# Autodesk Inventor assembly: Chassis assembly
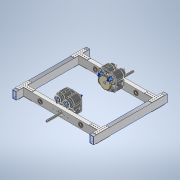
[picture p0: Inventor's stored thumbnail of the model, 180x180]
Saved by Autodesk Inventor 2022 (Build 260153000, 153)
## iProperties
Created: 2022-11-14
Part Number: Chassis assembly
Document SubType Name: Assembly
Designer: s135320
Author: s135320
## Documents named in this file (6)
- D:\Chassis assembly.iam
- D:\Chassis side 1.ipt
- D:\Chassis side 2.ipt
- D:\STEP Files\Hardware\Gussets\TTB T Gusset\TTB-00012_T-Gusset.ipt
- D:\STEP Files\Bearings\1-2inch Hex Bering\217-3875-STEP-20140818.ipt
- D:\STEP Files\Gearboxes\WCP SS Flipped Gearbox\WCP-0235.iam
## Components (22 placed, 5 different names)
1. Chassis side 1:1 — Mate:8, Mate:9, Flush:3, Mate:10, Mate:11, Flush:4, Mate:22, Mate:29, Mate:30, Mate:31, Mate:32, Mate:37, Mate:38, Mate:39, Mate:40, Mate:41, Mate:42, Mate:45
2. Chassis side 1:2 — Mate:1, Mate:2, Mate:3, Mate:14, Mate:15, Flush:6, Mate:16, Mate:17, Flush:7, Mate:20, Mate:25, Mate:26, Mate:27, Mate:28, Mate:33, Mate:34, Mate:35, Mate:36, Mate:43, Mate:44, Mate:46
3. Chassis side 2:1 — Mate:12, Mate:13, Flush:5, Mate:21, Flush:9, Mate:23, Mate:24
4. Chassis side 2:2 — Mate:4, Mate:5, Flush:1, Mate:6, Mate:7, Flush:2, Mate:18, Mate:19, Flush:8
5. TTB-00012_T-Gusset:1 — Mate:14, Mate:15, Flush:6
6. TTB-00012_T-Gusset:2 — Mate:1, Mate:2, Mate:3, Mate:4, Mate:5, Flush:1
7. TTB-00012_T-Gusset:3 — Mate:22, Mate:23, Mate:24
8. TTB-00012_T-Gusset:4 — Mate:16, Mate:17, Flush:7
9. TTB-00012_T-Gusset:5 — Mate:20, Mate:21, Flush:9
10. TTB-00012_T-Gusset:6 — Mate:6, Mate:7, Flush:2, Mate:8, Mate:9, Flush:3
11. TTB-00012_T-Gusset:7 — Mate:10, Mate:11, Flush:4, Mate:12, Mate:13, Flush:5
12. TTB-00012_T-Gusset:8 — Mate:18, Mate:19, Flush:8
13. 217-3875-STEP-20140818:3 — Mate:37, Mate:38
14. 217-3875-STEP-20140818:4 — Mate:29, Mate:30
15. 217-3875-STEP-20140818:5 — Mate:39, Mate:40
16. 217-3875-STEP-20140818:6 — Mate:35, Mate:36
17. 217-3875-STEP-20140818:8 — Mate:33, Mate:34
18. 217-3875-STEP-20140818:9 — Mate:31, Mate:32
19. 217-3875-STEP-20140818:11 — Mate:27, Mate:28
20. 217-3875-STEP-20140818:12 — Mate:25, Mate:26
21. WCP-0235:1 [sub-assembly] — Mate:43, Mate:44, Mate:46
22. WCP-0235:2 [sub-assembly] — Mate:41, Mate:42, Mate:45
## Relationships (55: Mate 46, Flush 9)
- Mate:1: Chassis side 1:2 ↔ TTB-00012_T-Gusset:2
- Mate:2: Chassis side 1:2 ↔ TTB-00012_T-Gusset:2
- Mate:3: Chassis side 1:2 ↔ TTB-00012_T-Gusset:2
- Mate:4: Chassis side 2:2 ↔ TTB-00012_T-Gusset:2
- Mate:5: Chassis side 2:2 ↔ TTB-00012_T-Gusset:2
- Flush:1: Chassis side 2:2 ↔ TTB-00012_T-Gusset:2
- Mate:6: Chassis side 2:2 ↔ TTB-00012_T-Gusset:6
- Mate:7: Chassis side 2:2 ↔ TTB-00012_T-Gusset:6
- Flush:2: Chassis side 2:2 ↔ TTB-00012_T-Gusset:6
- Mate:8: Chassis side 1:1 ↔ TTB-00012_T-Gusset:6
- Mate:9: Chassis side 1:1 ↔ TTB-00012_T-Gusset:6
- Flush:3: Chassis side 1:1 ↔ TTB-00012_T-Gusset:6
- Mate:10: Chassis side 1:1 ↔ TTB-00012_T-Gusset:7
- Mate:11: Chassis side 1:1 ↔ TTB-00012_T-Gusset:7
- Flush:4: Chassis side 1:1 ↔ TTB-00012_T-Gusset:7
- Mate:12: Chassis side 2:1 ↔ TTB-00012_T-Gusset:7
- Mate:13: Chassis side 2:1 ↔ TTB-00012_T-Gusset:7
- Flush:5: Chassis side 2:1 ↔ TTB-00012_T-Gusset:7
- Mate:14: Chassis side 1:2 ↔ TTB-00012_T-Gusset:1
- Mate:15: Chassis side 1:2 ↔ TTB-00012_T-Gusset:1
- Flush:6: Chassis side 1:2 ↔ TTB-00012_T-Gusset:1
- Mate:16: Chassis side 1:2 ↔ TTB-00012_T-Gusset:4
- Mate:17: Chassis side 1:2 ↔ TTB-00012_T-Gusset:4
- Flush:7: Chassis side 1:2 ↔ TTB-00012_T-Gusset:4
- Mate:18: Chassis side 2:2 ↔ TTB-00012_T-Gusset:8
- Mate:19: Chassis side 2:2 ↔ TTB-00012_T-Gusset:8
- Flush:8: Chassis side 2:2 ↔ TTB-00012_T-Gusset:8
- Mate:20: Chassis side 1:2 ↔ TTB-00012_T-Gusset:5
- Mate:21: Chassis side 2:1 ↔ TTB-00012_T-Gusset:5
- Flush:9: Chassis side 2:1 ↔ TTB-00012_T-Gusset:5
- Mate:22: Chassis side 1:1 ↔ TTB-00012_T-Gusset:3
- Mate:23: Chassis side 2:1 ↔ TTB-00012_T-Gusset:3
- Mate:24: Chassis side 2:1 ↔ TTB-00012_T-Gusset:3
- Mate:25: Chassis side 1:2 ↔ 217-3875-STEP-20140818:12
- Mate:26: Chassis side 1:2 ↔ 217-3875-STEP-20140818:12
- Mate:27: Chassis side 1:2 ↔ 217-3875-STEP-20140818:11
- Mate:28: Chassis side 1:2 ↔ 217-3875-STEP-20140818:11
- Mate:29: Chassis side 1:1 ↔ 217-3875-STEP-20140818:4
- Mate:30: Chassis side 1:1 ↔ 217-3875-STEP-20140818:4
- Mate:31: Chassis side 1:1 ↔ 217-3875-STEP-20140818:9
- Mate:32: Chassis side 1:1 ↔ 217-3875-STEP-20140818:9
- Mate:33: Chassis side 1:2 ↔ 217-3875-STEP-20140818:8
- Mate:34: Chassis side 1:2 ↔ 217-3875-STEP-20140818:8
- Mate:35: Chassis side 1:2 ↔ 217-3875-STEP-20140818:6
- Mate:36: Chassis side 1:2 ↔ 217-3875-STEP-20140818:6
- Mate:37: Chassis side 1:1 ↔ 217-3875-STEP-20140818:3
- Mate:38: Chassis side 1:1 ↔ 217-3875-STEP-20140818:3
- Mate:39: Chassis side 1:1 ↔ 217-3875-STEP-20140818:5
- Mate:40: Chassis side 1:1 ↔ 217-3875-STEP-20140818:5
- Mate:41: Chassis side 1:1 ↔ WCP-0235:2
- Mate:42: Chassis side 1:1 ↔ WCP-0235:2
- Mate:43: Chassis side 1:2 ↔ WCP-0235:1
- Mate:44: Chassis side 1:2 ↔ WCP-0235:1
- Mate:45: Chassis side 1:1 ↔ WCP-0235:2
- Mate:46: Chassis side 1:2 ↔ WCP-0235:1
